# Autodesk Inventor assembly: cellSTORM_v5
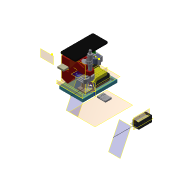
[picture p0: Inventor's stored thumbnail of the model, 180x180]
Saved by Autodesk Inventor 2019.4 (Build 234330000, 330)
## iProperties
Created: 2020-04-25
Part Number: cellSTORM_v5
Document SubType Name: Assembly
Designer: diederichbenedict
Author: diederichbenedict
## Documents named in this file (27)
- C:\Users\diederichbenedict\Dropbox\Dokumente\Promotion\PROJECTS\STORMoChip\GITHUB\CAD\Nanoscopy-on-the-cheap\Workspace\cellSTORM_v5.iam
- C:\Users\diederichbenedict\Dropbox\Dokumente\Promotion\PROJECTS\STORMoChip\GITHUB\CAD\Nanoscopy-on-the-cheap\Workspace\00_LASER_640nm.ipt
- C:\Users\diederichbenedict\Dropbox\Dokumente\Promotion\PROJECTS\STORMoChip\GITHUB\CAD\Nanoscopy-on-the-cheap\Workspace\00_XY_stage-CHUO_SEIKI_LD-647-R1.iam
- C:\Users\diederichbenedict\Dropbox\Dokumente\Promotion\PROJECTS\STORMoChip\GITHUB\CAD\Nanoscopy-on-the-cheap\Workspace\cellSTORM_laserbeam.ipt
- C:\Users\diederichbenedict\Dropbox\Dokumente\Promotion\PROJECTS\STORMoChip\GITHUB\CAD\Nanoscopy-on-the-cheap\Workspace\02_Nanoscopy_Chip.ipt
- C:\Users\diederichbenedict\Dropbox\Dokumente\Promotion\PROJECTS\STORMoChip\GITHUB\CAD\Nanoscopy-on-the-cheap\Workspace\cellSTORM_nickelplate.ipt
- C:\Users\diederichbenedict\Dropbox\Dokumente\Promotion\PROJECTS\STORMoChip\GITHUB\CAD\Nanoscopy-on-the-cheap\Workspace\00_Ballmagnets_5mm.ipt
- C:\Users\diederichbenedict\Documents\Inventor\Content Center Files\R2019\en-US\DIN 912\DIN 912 - M3 x 0.5 x 25 x 18.ipt
- C:\Users\diederichbenedict\Dropbox\Dokumente\Promotion\PROJECTS\STORMoChip\GITHUB\CAD\Nanoscopy-on-the-cheap\Workspace\00_Huawei_P20.ipt
- C:\Users\diederichbenedict\Dropbox\Dokumente\Promotion\PROJECTS\STORMoChip\GITHUB\CAD\Nanoscopy-on-the-cheap\Workspace\cellSTORM_Base_v0_R1.ipt
- C:\Users\diederichbenedict\Dropbox\Dokumente\Promotion\PROJECTS\STORMoChip\GITHUB\CAD\Nanoscopy-on-the-cheap\Workspace\00_KES400.iam
- C:\Users\diederichbenedict\Dropbox\Dokumente\Promotion\PROJECTS\STORMoChip\GITHUB\CAD\Nanoscopy-on-the-cheap\Workspace\cellSTORM_v5_laserstage.ipt
- C:\Users\diederichbenedict\Dropbox\Dokumente\Promotion\PROJECTS\STORMoChip\GITHUB\CAD\Nanoscopy-on-the-cheap\Workspace\cellSTORM_v5_cellphonestage.ipt
- C:\Users\diederichbenedict\Dropbox\Dokumente\Promotion\PROJECTS\STORMoChip\GITHUB\CAD\Nanoscopy-on-the-cheap\Workspace\cellSTORM_v5_microsocpe.iam
- C:\Users\diederichbenedict\Dropbox\Dokumente\Promotion\PROJECTS\STORMoChip\GITHUB\CAD\Nanoscopy-on-the-cheap\Workspace\cellSTORM_v5_microscope_cover.ipt
- C:\Users\diederichbenedict\Dropbox\Dokumente\Promotion\PROJECTS\STORMoChip\GITHUB\CAD\Nanoscopy-on-the-cheap\Workspace\00_Stepper_Motor_28BYJ-48.0013.ipt
- C:\Users\diederichbenedict\Dropbox\Dokumente\Promotion\PROJECTS\STORMoChip\GITHUB\CAD\Nanoscopy-on-the-cheap\Workspace\cellSTORM_v5_focusmotormount.ipt
- C:\Users\diederichbenedict\Dropbox\Dokumente\Promotion\PROJECTS\STORMoChip\GITHUB\CAD\Nanoscopy-on-the-cheap\Workspace\Raspi\BD-DRIVE_PULLEY.ipt
- C:\Users\diederichbenedict\Dropbox\Dokumente\Promotion\PROJECTS\STORMoChip\GITHUB\CAD\Nanoscopy-on-the-cheap\Workspace\cellSTORM_focusmotor_pulley.ipt
- C:\Users\diederichbenedict\Dropbox\Dokumente\Promotion\PROJECTS\STORMoChip\GITHUB\CAD\Nanoscopy-on-the-cheap\Workspace\cellSTORM_v5_ELECTRONICS.iam
- C:\Users\diederichbenedict\Dropbox\Dokumente\Promotion\PROJECTS\STORMoChip\GITHUB\CAD\Nanoscopy-on-the-cheap\Workspace\00_chip_01_old.ipt
- C:\Users\diederichbenedict\Dropbox\Dokumente\Promotion\PROJECTS\STORMoChip\GITHUB\CAD\Nanoscopy-on-the-cheap\Workspace\cellSTORM_v5_chiptray_old_0.ipt
- C:\Users\diederichbenedict\Dropbox\Dokumente\Promotion\PROJECTS\STORMoChip\GITHUB\CAD\Nanoscopy-on-the-cheap\Workspace\cellSTORM_v5_chiptry_clamp.ipt
- C:\Users\diederichbenedict\Dropbox\Dokumente\Promotion\PROJECTS\STORMoChip\GITHUB\CAD\Nanoscopy-on-the-cheap\Workspace\00_chip_01_new.ipt
- C:\Users\diederichbenedict\Dropbox\Dokumente\Promotion\PROJECTS\STORMoChip\GITHUB\CAD\Nanoscopy-on-the-cheap\Workspace\cellSTORM_v5_chiptray_new_0.ipt
- C:\Users\diederichbenedict\Dropbox\Dokumente\Promotion\PROJECTS\STORMoChip\GITHUB\CAD\Nanoscopy-on-the-cheap\Workspace\00_Laser_532nm_200mw.ipt
- C:\Users\diederichbenedict\Dropbox\Dokumente\Promotion\PROJECTS\STORMoChip\GITHUB\CAD\Nanoscopy-on-the-cheap\Workspace\cellSTORM_v5_laser_532nm_adapter.ipt
## Components (32 placed, 26 different names)
1. 00_LASER_640nm:1 — Insert:2, Angle:6, Mate:7, Mate:6, Flush:1, Angle:7, Flush:27
2. 00_XY_stage-CHUO_SEIKI_LD-647-R1:1 [sub-assembly] — Insert:1, Angle:1, Insert:6, Angle:5, Mate:6, Flush:1, Flush:10, Flush:11
3. cellSTORM_laserbeam:1 — Insert:2, Insert:3, Insert:7, Insert:16, Mate:27
4. 02_Nanoscopy_Chip:1 — Insert:3, Angle:2, Mate:9, Mate:11
5. cellSTORM_nickelplate:1 — Mate:9
6. 00_Ballmagnets_5mm:1
7. DIN 912 - replaced by DIN EN ISO 4762 M3 x 25:1 — Insert:4
8. 00_Ballmagnets_5mm:2
9. DIN 912 - replaced by DIN EN ISO 4762 M3 x 25:2 — Insert:13
10. 00_Ballmagnets_5mm:3
11. DIN 912 - replaced by DIN EN ISO 4762 M3 x 25:3 — Insert:14
12. cellSTORM_Base_v0_R1:1 — Insert:1, Angle:1, Angle:2, Insert:4, Angle:6, Mate:7, Insert:13, Insert:14, Flush:23
13. 00_XY_stage-CHUO_SEIKI_LD-647-R1:2 [sub-assembly] — Insert:6, Angle:5, Flush:12, Flush:13
14. 00_KES400:1 [sub-assembly] — Insert:7, Angle:7, Mate:27, Mate:28
15. cellSTORM_v5_laserstage:1 — Flush:10, Flush:11
16. cellSTORM_v5_cellphonestage:1 — Flush:12, Flush:13, Mate:10, Flush:14, Flush:17, Flush:18, Flush:19, Mate:24
17. cellSTORM_v5_microsocpe:1 [sub-assembly] — Mate:10, Mate:11, Flush:14, Flush:15, Flush:16, Mate:18, Mate:19, Mate:20, Mate:23
18. cellSTORM_v5_microscope_cover:1 — Flush:15, Flush:16
19. 00_Stepper_Motor_28BYJ-48.0013:1 — Mate:18, Mate:19, Flush:17, Flush:20, Insert:15
20. cellSTORM_v5_focusmotormount:1 — Flush:18, Flush:19, Flush:20
21. BD-DRIVE_PULLEY:1 — Insert:15, Flush:21
22. cellSTORM_focusmotor_pulley:1 — Mate:20, Flush:21
23. 00_Huawei_P20:1 — Mate:23, Mate:24
24. cellSTORM_v5_ELECTRONICS:1 [sub-assembly]
25. 00_chip_01_old:1 — Flush:22, Insert:16
26. cellSTORM_v5_chiptray_old_0:1 — Flush:22, Flush:23, Flush:24, Flush:25
27. cellSTORM_v5_chiptry_clamp:1 — Flush:24, Flush:25
28. 00_chip_01_new:1 — Mate:25, Mate:26, Flush:26
29. cellSTORM_v5_chiptray_new_0:1 — Mate:25, Mate:26, Flush:26
30. 00_Laser_532nm_200mw:1 — Mate:28, Flush:27, Flush:28
31. cellSTORM_v5_laser_532nm_adapter:1 — Flush:28, Flush:29
32. 00_Laser_532nm_200mw:2 — Flush:29
## Relationships (54: Flush 21, Mate 18, Insert 10, Angle 5)
- [Mate]: 02_Nanoscopy_Chip:1 ↔ cellSTORM_nickelplate:1
- [Mate]: 00_Ballmagnets_5mm:1 ↔ DIN 912 - replaced by DIN EN ISO 4762 M3 x 25:1
- [Mate]: 00_Ballmagnets_5mm:2 ↔ DIN 912 - replaced by DIN EN ISO 4762 M3 x 25:2
- [Mate]: 00_Ballmagnets_5mm:3 ↔ DIN 912 - replaced by DIN EN ISO 4762 M3 x 25:3
- Insert:1: 00_XY_stage-CHUO_SEIKI_LD-647-R1:1 ↔ cellSTORM_Base_v0_R1:1
- Angle:1 (90 deg): 00_XY_stage-CHUO_SEIKI_LD-647-R1:1 ↔ cellSTORM_Base_v0_R1:1
- Insert:2 (-10 mm): 00_LASER_640nm:1 ↔ cellSTORM_laserbeam:1
- Insert:3 (5 mm): cellSTORM_laserbeam:1 ↔ 02_Nanoscopy_Chip:1
- Angle:2 (180 deg): 02_Nanoscopy_Chip:1 ↔ cellSTORM_Base_v0_R1:1
- Insert:4 (-15 mm): DIN 912 - replaced by DIN EN ISO 4762 M3 x 25:1 ↔ cellSTORM_Base_v0_R1:1
- Insert:6 (6 mm): 00_XY_stage-CHUO_SEIKI_LD-647-R1:1 ↔ 00_XY_stage-CHUO_SEIKI_LD-647-R1:2
- Angle:5 (180 deg): 00_XY_stage-CHUO_SEIKI_LD-647-R1:1 ↔ 00_XY_stage-CHUO_SEIKI_LD-647-R1:2
- Angle:6 (0 deg): 00_LASER_640nm:1 ↔ cellSTORM_Base_v0_R1:1
- Mate:7 (1 mm): 00_LASER_640nm:1 ↔ cellSTORM_Base_v0_R1:1
- Mate:6 (10 mm): 00_LASER_640nm:1 ↔ 00_XY_stage-CHUO_SEIKI_LD-647-R1:1
- Flush:1 (-5 mm): 00_LASER_640nm:1 ↔ 00_XY_stage-CHUO_SEIKI_LD-647-R1:1
- Insert:7: cellSTORM_laserbeam:1 ↔ 00_KES400:1
- Angle:7 (0 deg): 00_LASER_640nm:1 ↔ 00_KES400:1
- Insert:13 (-15 mm): DIN 912 - replaced by DIN EN ISO 4762 M3 x 25:2 ↔ cellSTORM_Base_v0_R1:1
- Insert:14 (-15 mm): DIN 912 - replaced by DIN EN ISO 4762 M3 x 25:3 ↔ cellSTORM_Base_v0_R1:1
- Mate:9: 02_Nanoscopy_Chip:1 ↔ cellSTORM_nickelplate:1
- Flush:10: 00_XY_stage-CHUO_SEIKI_LD-647-R1:1 ↔ cellSTORM_v5_laserstage:1
- Flush:11: 00_XY_stage-CHUO_SEIKI_LD-647-R1:1 ↔ cellSTORM_v5_laserstage:1
- Flush:12: 00_XY_stage-CHUO_SEIKI_LD-647-R1:2 ↔ cellSTORM_v5_cellphonestage:1
- Flush:13: 00_XY_stage-CHUO_SEIKI_LD-647-R1:2 ↔ cellSTORM_v5_cellphonestage:1
- Mate:10: cellSTORM_v5_cellphonestage:1 ↔ cellSTORM_v5_microsocpe:1
- Mate:11: 02_Nanoscopy_Chip:1 ↔ cellSTORM_v5_microsocpe:1
- Flush:14: cellSTORM_v5_cellphonestage:1 ↔ cellSTORM_v5_microsocpe:1
- Flush:15: cellSTORM_v5_microsocpe:1 ↔ cellSTORM_v5_microscope_cover:1
- Flush:16: cellSTORM_v5_microsocpe:1 ↔ cellSTORM_v5_microscope_cover:1
- Mate:18 (10 mm): cellSTORM_v5_microsocpe:1 ↔ 00_Stepper_Motor_28BYJ-48.0013:1
- Mate:19 (35 mm): cellSTORM_v5_microsocpe:1 ↔ 00_Stepper_Motor_28BYJ-48.0013:1
- Flush:17 (-40 mm): cellSTORM_v5_cellphonestage:1 ↔ 00_Stepper_Motor_28BYJ-48.0013:1
- Flush:18: cellSTORM_v5_cellphonestage:1 ↔ cellSTORM_v5_focusmotormount:1
- Flush:19: cellSTORM_v5_cellphonestage:1 ↔ cellSTORM_v5_focusmotormount:1
- Flush:20: 00_Stepper_Motor_28BYJ-48.0013:1 ↔ cellSTORM_v5_focusmotormount:1
- Insert:15: 00_Stepper_Motor_28BYJ-48.0013:1 ↔ BD-DRIVE_PULLEY:1
- Mate:20: cellSTORM_v5_microsocpe:1 ↔ cellSTORM_focusmotor_pulley:1
- Flush:21: BD-DRIVE_PULLEY:1 ↔ cellSTORM_focusmotor_pulley:1
- Mate:23: cellSTORM_v5_microsocpe:1 ↔ 00_Huawei_P20:1
- Mate:24: cellSTORM_v5_cellphonestage:1 ↔ 00_Huawei_P20:1
- Flush:22: 00_chip_01_old:1 ↔ cellSTORM_v5_chiptray_old_0:1
- Flush:23 (10 mm): cellSTORM_Base_v0_R1:1 ↔ cellSTORM_v5_chiptray_old_0:1
- Insert:16: cellSTORM_laserbeam:1 ↔ 00_chip_01_old:1
- Flush:24: cellSTORM_v5_chiptray_old_0:1 ↔ cellSTORM_v5_chiptry_clamp:1
- Flush:25: cellSTORM_v5_chiptray_old_0:1 ↔ cellSTORM_v5_chiptry_clamp:1
- Mate:25: 00_chip_01_new:1 ↔ cellSTORM_v5_chiptray_new_0:1
- Mate:26: 00_chip_01_new:1 ↔ cellSTORM_v5_chiptray_new_0:1
- Flush:26 (-3 mm): 00_chip_01_new:1 ↔ cellSTORM_v5_chiptray_new_0:1
- Mate:27: cellSTORM_laserbeam:1 ↔ 00_KES400:1
- Mate:28: 00_KES400:1 ↔ 00_Laser_532nm_200mw:1
- Flush:27: 00_LASER_640nm:1 ↔ 00_Laser_532nm_200mw:1
- Flush:28: 00_Laser_532nm_200mw:1 ↔ cellSTORM_v5_laser_532nm_adapter:1
- Flush:29: cellSTORM_v5_laser_532nm_adapter:1 ↔ 00_Laser_532nm_200mw:2
## Named parameters: d2_d162 = 0 mm, d3_d162 = 0 mm
